# Autodesk Inventor assembly: Złożenie całości
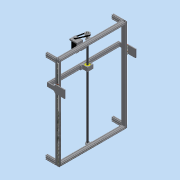
[picture p0: Inventor's stored thumbnail of the model, 180x180]
Saved by Autodesk Inventor 2018 (Build 220112000, 112)
## iProperties
Created: 2019-01-23
Part Number: Złożenie całości
Material: Ogólny
Document SubType Name: Assembly
Designer: Dawid
Author: Dawid
## Documents named in this file (24)
- E:\Frezarka_K2\INVENTOR\ZŁOŻENIA\Złożenie całości.iam
- E:\Frezarka_K2\INVENTOR\RAMA\Profil dolny długi.ipt
- E:\Frezarka_K2\INVENTOR\RAMA\Profil dolny krótki.ipt
- E:\Frezarka_K2\INVENTOR\RAMA\Profil dolny - noga.ipt
- E:\Frezarka_K2\INVENTOR\NAPĘD\Śruba trapezowa 16x4.ipt
- E:\Frezarka_K2\INVENTOR\NAPĘD\Łożysko w obudowie aluminiowej 10mm KP000.ipt
- C:\Users\Dawid\Documents\Inventor\Content Center Files\R2018\pl-PL\DIN 6926\DIN 6926 - M10 x 1,5.ipt
- E:\Frezarka_K2\INVENTOR\NAPĘD\Koło zębate 21 T5 28 2F.ipt
- E:\Frezarka_K2\INVENTOR\NAPĘD\Tuleja zaciskowo rozprężna RCK BK 80 8x15 Clampex.ipt
- C:\Users\Dawid\Documents\Inventor\Content Center Files\R2018\pl-PL\CNS 3932\CNS 3932 - M 4 x 0,7 x 6.ipt
- E:\Frezarka_K2\INVENTOR\NAPĘD\Silnik krokowy SM 60 100-4004AF - 4Nm.ipt
- E:\Frezarka_K2\INVENTOR\NAPĘD\Koło zębate 21 T5 14 2F.ipt
- E:\Frezarka_K2\INVENTOR\NAPĘD\Uchwyt silnika krokowego osi Y.ipt
- C:\Users\Dawid\Documents\Inventor\Content Center Files\R2018\pl-PL\CNS 3932\CNS 3932 - M 5 x 0,8 x 12.ipt
- E:\Frezarka_K2\INVENTOR\NAPĘD\Pas zębaty 10 T5-315.ipt
- C:\Users\Dawid\Documents\Inventor\Content Center Files\R2018\pl-PL\CNS 3932\CNS 3932 - M 5 x 0,8 x 10.ipt
- E:\Frezarka_K2\INVENTOR\NAPĘD\Nakrętka trapezowa kołnierzowa JFRM-2835TR16x4.ipt
- E:\Frezarka_K2\INVENTOR\NAPĘD\Obudowa nakrętki trapezowej fi 16.ipt
- E:\Frezarka_K2\INVENTOR\RAMA\Profil dolny posuwu osi Y.ipt
- E:\Frezarka_K2\INVENTOR\NAPĘD\Prowadnica liniowa MGN9R 900mm.ipt
- E:\Frezarka_K2\INVENTOR\NAPĘD\Wózek MGN9C.ipt
- E:\Frezarka_K2\INVENTOR\NAPĘD\Wspornik pionowy osi Y.ipt
- C:\Users\Dawid\Documents\Inventor\Content Center Files\R2018\pl-PL\CNS 3932\CNS 3932 - M 3 x 0,5 x 5.ipt
- E:\Frezarka_K2\INVENTOR\RAMA\Sklejka stołu.ipt
## Components (82 placed, 23 different names)
1. Profil dolny długi:1 — Zestawiający:1, Zestawiający:4, Równoległy:19, Równoległy:20, Zestawiający:35, Zestawiający:40, Równoległy:28, Równoległy:29, Zestawiający:41, Równoległy:30, Równoległy:31, Zestawiający:44, Równoległy:36, Równoległy:43, Równoległy:44, Równoległy:45
2. Profil dolny krótki:1 — Zestawiający:1, Zestawiający:2, Równoległy:23, Równoległy:24, Zestawiający:38, Zestawiający:61, Równoległy:49
3. Profil dolny długi:2 — Zestawiający:2, Zestawiający:3, Zestawiający:5, Zestawiający:6, Zestawiający:20, Równoległy:21, Równoległy:22, Równoległy:23, Równoległy:24, Zestawiający:39, Równoległy:26, Równoległy:27, Zestawiający:42, Równoległy:32, Równoległy:33, Zestawiający:45, Równoległy:38, Równoległy:48
4. Profil dolny krótki:2 — Zestawiający:3, Równoległy:19, Równoległy:20, Równoległy:21, Równoległy:22, Zestawiający:34, Równoległy:25, Zestawiający:36, Zestawiający:37, Równoległy:37, Równoległy:39
5. Profil dolny - noga:1 — Zestawiający:5, Zestawiający:42, Równoległy:32, Równoległy:33
6. Profil dolny - noga:2 — Zestawiający:6, Zestawiający:39, Równoległy:26, Równoległy:27
7. Profil dolny - noga:3 — Zestawiający:41, Równoległy:30, Równoległy:31
8. Profil dolny - noga:4 — Zestawiający:4, Zestawiający:40, Równoległy:28, Równoległy:29
9. Śruba trapezowa 16x4:1 — Zestawiający:8, Zestawiający:9, Zestawiający:10, Zestawiający:11, Zestawiający:12, Zestawiający:18, Zestawiający:19, Zestawiający:31
10. Łożysko w obudowie aluminiowej 10mm KP000:1 — Zestawiający:8, Zestawiający:9, Zestawiający:13, Zestawiający:20, Zestawiający:34, Zestawiający:35, Równoległy:25
11. Łożysko w obudowie aluminiowej 10mm KP000:2 — Zestawiający:10, Zestawiający:11, Zestawiający:38
12. DIN 6926 - zastąpiona przez DIN EN 1663/1666 M10:1 — Zestawiający:12, Zestawiający:13
13. Koło zębate 21 T5 28 2F:1 — Zestawiający:16, Zestawiający:17, Zestawiający:28
14. Tuleja zaciskowo rozprężna RCK BK 80 8x15 Clampex:1 — Zestawiający:16, Zestawiający:17, Zestawiający:18, Zestawiający:19, Wstaw:1, Wstaw:2, Wstaw:3, Wstaw:4, Wstaw:5, Wstaw:6
15. CNS 3932 M 4 x 6:1 — Wstaw:1
16. CNS 3932 M 4 x 6:2 — Wstaw:2
17. CNS 3932 M 4 x 6:3 — Wstaw:3
18. CNS 3932 M 4 x 6:4 — Wstaw:4
19. CNS 3932 M 4 x 6:5 — Wstaw:5
20. CNS 3932 M 4 x 6:6 — Wstaw:6
21. Silnik krokowy SM 60 100-4004AF - 4Nm:1 — Zestawiający:21, Zestawiający:22, Zestawiający:23, Zestawiający:24, Zestawiający:25, Wstaw:7, Wstaw:8, Wstaw:9, Wstaw:10
22. Koło zębate 21 T5 14 2F:1 — Zestawiający:21, Zestawiający:22, Zestawiający:29
23. Uchwyt silnika krokowego osi Y:1 — Zestawiający:23, Zestawiający:24, Zestawiający:25, Wstaw:11, Wstaw:12, Wstaw:13, Wstaw:14, Zestawiający:36, Zestawiający:37
24. CNS 3932 M 5 x 12:1 — Wstaw:7
25. CNS 3932 M 5 x 12:2 — Wstaw:8
26. CNS 3932 M 5 x 12:3 — Wstaw:9
27. CNS 3932 M 5 x 12:4 — Wstaw:10
28. Pas zębaty 10 T5-315:1 — Zestawiający:28, Zestawiający:29
29. CNS 3932 M 5 x 10:1 — Wstaw:11
30. CNS 3932 M 5 x 10:2 — Wstaw:12
31. CNS 3932 M 5 x 10:3 — Wstaw:13
32. CNS 3932 M 5 x 10:4 — Wstaw:14
33. Nakrętka trapezowa kołnierzowa JFRM-2835TR16x4:1 — Zestawiający:31, Zestawiający:32, Zestawiający:33
34. Obudowa nakrętki trapezowej fi 16:1 — Zestawiający:32, Zestawiający:33, Równoległy:18, Zestawiający:43, Równoległy:34, Równoległy:35
35. Profil dolny posuwu osi Y:1 — Równoległy:18, Zestawiający:43, Równoległy:34, Równoległy:35, Równoległy:40, Zestawiający:54, Równoległy:41, Równoległy:42, Zestawiający:58, Równoległy:46, Równoległy:47
36. Prowadnica liniowa MGN9R 900mm:1 — Zestawiający:44, Równoległy:36, Równoległy:37, Zestawiający:50, Zestawiający:51, Zestawiający:52, Zestawiający:53, Wstaw:34, Wstaw:35, Wstaw:36, Wstaw:37, Wstaw:38, Wstaw:39, Wstaw:40, Wstaw:41, Wstaw:42, Wstaw:43, Wstaw:44, Wstaw:45, Wstaw:46, Wstaw:47, Wstaw:48, Wstaw:49, Wstaw:50, Wstaw:51, Wstaw:52
37. Prowadnica liniowa MGN9R 900mm:2 — Zestawiający:45, Równoległy:38, Równoległy:39, Zestawiający:46, Zestawiający:47, Zestawiający:48, Zestawiający:49, Zestawiający:57, Wstaw:15, Wstaw:16, Wstaw:17, Wstaw:18, Wstaw:19, Wstaw:20, Wstaw:21, Wstaw:22, Wstaw:23, Wstaw:24, Wstaw:25, Wstaw:26, Wstaw:27, Wstaw:28, Wstaw:29, Wstaw:30, Wstaw:31, Wstaw:32, Wstaw:33
38. Wózek MGN9C:1 — Zestawiający:46, Zestawiający:47, Zestawiający:59
39. Wózek MGN9C:2 — Zestawiający:48, Zestawiający:49, Zestawiający:57, Zestawiający:60
40. Wózek MGN9C:3 — Zestawiający:50, Zestawiający:51, Zestawiający:55
41. Wózek MGN9C:4 — Zestawiający:52, Zestawiający:53, Równoległy:40, Zestawiający:56
42. Wspornik pionowy osi Y:1 — Zestawiający:54, Równoległy:41, Równoległy:42, Zestawiający:55, Zestawiający:56
43. Wspornik pionowy osi Y:2 — Zestawiający:58, Równoległy:46, Równoległy:47, Zestawiający:59, Zestawiający:60
44. CNS 3932 M 3 x 5:1 — Wstaw:15
45. CNS 3932 M 3 x 5:2 — Wstaw:16
46. CNS 3932 M 3 x 5:3 — Wstaw:17
47. CNS 3932 M 3 x 5:4 — Wstaw:18
48. CNS 3932 M 3 x 5:5 — Wstaw:19
49. CNS 3932 M 3 x 5:6 — Wstaw:20
50. CNS 3932 M 3 x 5:7 — Wstaw:21
51. CNS 3932 M 3 x 5:8 — Wstaw:22
52. CNS 3932 M 3 x 5:9 — Wstaw:23
53. CNS 3932 M 3 x 5:10 — Wstaw:24
54. CNS 3932 M 3 x 5:11 — Wstaw:25
55. CNS 3932 M 3 x 5:12 — Wstaw:26
56. CNS 3932 M 3 x 5:13 — Wstaw:27
57. CNS 3932 M 3 x 5:14 — Wstaw:28
58. CNS 3932 M 3 x 5:15 — Wstaw:29
59. CNS 3932 M 3 x 5:16 — Wstaw:30
60. CNS 3932 M 3 x 5:17 — Wstaw:31
61. CNS 3932 M 3 x 5:18 — Wstaw:32
62. CNS 3932 M 3 x 5:19 — Wstaw:33
63. CNS 3932 M 3 x 5:20 — Wstaw:34
64. CNS 3932 M 3 x 5:21 — Wstaw:35
65. CNS 3932 M 3 x 5:22 — Wstaw:36
66. CNS 3932 M 3 x 5:23 — Wstaw:37
67. CNS 3932 M 3 x 5:24 — Wstaw:38
68. CNS 3932 M 3 x 5:25 — Wstaw:39
69. CNS 3932 M 3 x 5:26 — Wstaw:40
70. CNS 3932 M 3 x 5:27 — Wstaw:41
71. CNS 3932 M 3 x 5:28 — Wstaw:42
72. CNS 3932 M 3 x 5:29 — Wstaw:43
73. CNS 3932 M 3 x 5:30 — Wstaw:44
74. CNS 3932 M 3 x 5:31 — Wstaw:45
75. CNS 3932 M 3 x 5:32 — Wstaw:46
76. CNS 3932 M 3 x 5:33 — Wstaw:47
77. CNS 3932 M 3 x 5:34 — Wstaw:48
78. CNS 3932 M 3 x 5:35 — Wstaw:49
79. CNS 3932 M 3 x 5:36 — Wstaw:50
80. CNS 3932 M 3 x 5:37 — Wstaw:51
81. CNS 3932 M 3 x 5:38 — Wstaw:52
82. Sklejka stołu:1 — Zestawiający:61, Równoległy:48, Równoległy:49
## Relationships (139: Mate 55, Insert 52, Flush 32)
- Zestawiający:1 [Mate]: Profil dolny długi:1 ↔ Profil dolny krótki:1
- Zestawiający:2 [Mate]: Profil dolny krótki:1 ↔ Profil dolny długi:2
- Zestawiający:3 [Mate]: Profil dolny długi:2 ↔ Profil dolny krótki:2
- Zestawiający:4 [Mate]: Profil dolny długi:1 ↔ Profil dolny - noga:4
- Zestawiający:5 [Mate]: Profil dolny długi:2 ↔ Profil dolny - noga:1
- Zestawiający:6 [Mate]: Profil dolny długi:2 ↔ Profil dolny - noga:2
- Zestawiający:8 [Mate]: Śruba trapezowa 16x4:1 ↔ Łożysko w obudowie aluminiowej 10mm KP000:1
- Zestawiający:9 [Mate]: Śruba trapezowa 16x4:1 ↔ Łożysko w obudowie aluminiowej 10mm KP000:1
- Zestawiający:10 [Mate]: Śruba trapezowa 16x4:1 ↔ Łożysko w obudowie aluminiowej 10mm KP000:2
- Zestawiający:11 [Mate] (2 mm): Śruba trapezowa 16x4:1 ↔ Łożysko w obudowie aluminiowej 10mm KP000:2
- Zestawiający:12 [Mate]: Śruba trapezowa 16x4:1 ↔ DIN 6926 - zastąpiona przez DIN EN 1663/1666 M10:1
- Zestawiający:13 [Mate]: Łożysko w obudowie aluminiowej 10mm KP000:1 ↔ DIN 6926 - zastąpiona przez DIN EN 1663/1666 M10:1
- Zestawiający:16 [Mate]: Koło zębate 21 T5 28 2F:1 ↔ Tuleja zaciskowo rozprężna RCK BK 80 8x15 Clampex:1
- Zestawiający:17 [Mate]: Koło zębate 21 T5 28 2F:1 ↔ Tuleja zaciskowo rozprężna RCK BK 80 8x15 Clampex:1
- Zestawiający:18 [Mate]: Śruba trapezowa 16x4:1 ↔ Tuleja zaciskowo rozprężna RCK BK 80 8x15 Clampex:1
- Zestawiający:19 [Mate] (2 mm): Śruba trapezowa 16x4:1 ↔ Tuleja zaciskowo rozprężna RCK BK 80 8x15 Clampex:1
- Wstaw:1 [Insert]: Tuleja zaciskowo rozprężna RCK BK 80 8x15 Clampex:1 ↔ CNS 3932 M 4 x 6:1
- Wstaw:2 [Insert]: Tuleja zaciskowo rozprężna RCK BK 80 8x15 Clampex:1 ↔ CNS 3932 M 4 x 6:2
- Wstaw:3 [Insert]: Tuleja zaciskowo rozprężna RCK BK 80 8x15 Clampex:1 ↔ CNS 3932 M 4 x 6:3
- Wstaw:4 [Insert]: Tuleja zaciskowo rozprężna RCK BK 80 8x15 Clampex:1 ↔ CNS 3932 M 4 x 6:4
- Wstaw:5 [Insert]: Tuleja zaciskowo rozprężna RCK BK 80 8x15 Clampex:1 ↔ CNS 3932 M 4 x 6:5
- Wstaw:6 [Insert]: Tuleja zaciskowo rozprężna RCK BK 80 8x15 Clampex:1 ↔ CNS 3932 M 4 x 6:6
- Zestawiający:20 [Mate] (296.5 mm): Profil dolny długi:2 ↔ Łożysko w obudowie aluminiowej 10mm KP000:1
- Zestawiający:21 [Mate]: Silnik krokowy SM 60 100-4004AF - 4Nm:1 ↔ Koło zębate 21 T5 14 2F:1
- Zestawiający:22 [Mate] (1 mm): Silnik krokowy SM 60 100-4004AF - 4Nm:1 ↔ Koło zębate 21 T5 14 2F:1
- Zestawiający:23 [Mate]: Silnik krokowy SM 60 100-4004AF - 4Nm:1 ↔ Uchwyt silnika krokowego osi Y:1
- Zestawiający:24 [Mate]: Silnik krokowy SM 60 100-4004AF - 4Nm:1 ↔ Uchwyt silnika krokowego osi Y:1
- Zestawiający:25 [Mate]: Silnik krokowy SM 60 100-4004AF - 4Nm:1 ↔ Uchwyt silnika krokowego osi Y:1
- Wstaw:7 [Insert]: Silnik krokowy SM 60 100-4004AF - 4Nm:1 ↔ CNS 3932 M 5 x 12:1
- Wstaw:8 [Insert]: Silnik krokowy SM 60 100-4004AF - 4Nm:1 ↔ CNS 3932 M 5 x 12:2
- Wstaw:9 [Insert]: Silnik krokowy SM 60 100-4004AF - 4Nm:1 ↔ CNS 3932 M 5 x 12:3
- Wstaw:10 [Insert]: Silnik krokowy SM 60 100-4004AF - 4Nm:1 ↔ CNS 3932 M 5 x 12:4
- Zestawiający:28 [Mate]: Koło zębate 21 T5 28 2F:1 ↔ Pas zębaty 10 T5-315:1
- Zestawiający:29 [Mate]: Koło zębate 21 T5 14 2F:1 ↔ Pas zębaty 10 T5-315:1
- Wstaw:11 [Insert]: Uchwyt silnika krokowego osi Y:1 ↔ CNS 3932 M 5 x 10:1
- Wstaw:12 [Insert]: Uchwyt silnika krokowego osi Y:1 ↔ CNS 3932 M 5 x 10:2
- Wstaw:13 [Insert]: Uchwyt silnika krokowego osi Y:1 ↔ CNS 3932 M 5 x 10:3
- Wstaw:14 [Insert]: Uchwyt silnika krokowego osi Y:1 ↔ CNS 3932 M 5 x 10:4
- Zestawiający:31 [Mate]: Śruba trapezowa 16x4:1 ↔ Nakrętka trapezowa kołnierzowa JFRM-2835TR16x4:1
- Zestawiający:32 [Mate]: Nakrętka trapezowa kołnierzowa JFRM-2835TR16x4:1 ↔ Obudowa nakrętki trapezowej fi 16:1
- Zestawiający:33 [Mate]: Nakrętka trapezowa kołnierzowa JFRM-2835TR16x4:1 ↔ Obudowa nakrętki trapezowej fi 16:1
- Równoległy:18 [Flush] (310 mm): Obudowa nakrętki trapezowej fi 16:1 ↔ Profil dolny posuwu osi Y:1
- Równoległy:19 [Flush]: Profil dolny długi:1 ↔ Profil dolny krótki:2
- Równoległy:20 [Flush]: Profil dolny długi:1 ↔ Profil dolny krótki:2
- Równoległy:21 [Flush]: Profil dolny długi:2 ↔ Profil dolny krótki:2
- Równoległy:22 [Flush]: Profil dolny długi:2 ↔ Profil dolny krótki:2
- Równoległy:23 [Flush]: Profil dolny krótki:1 ↔ Profil dolny długi:2
- Równoległy:24 [Flush]: Profil dolny krótki:1 ↔ Profil dolny długi:2
- Zestawiający:34 [Mate]: Profil dolny krótki:2 ↔ Łożysko w obudowie aluminiowej 10mm KP000:1
- Zestawiający:35 [Mate] (296.5 mm): Profil dolny długi:1 ↔ Łożysko w obudowie aluminiowej 10mm KP000:1
- Równoległy:25 [Flush] (2 mm): Profil dolny krótki:2 ↔ Łożysko w obudowie aluminiowej 10mm KP000:1
- Zestawiający:36 [Mate]: Profil dolny krótki:2 ↔ Uchwyt silnika krokowego osi Y:1
- Zestawiający:37 [Mate]: Profil dolny krótki:2 ↔ Uchwyt silnika krokowego osi Y:1
- Zestawiający:38 [Mate]: Profil dolny krótki:1 ↔ Łożysko w obudowie aluminiowej 10mm KP000:2
- Zestawiający:39 [Mate]: Profil dolny długi:2 ↔ Profil dolny - noga:2
- Równoległy:26 [Flush]: Profil dolny długi:2 ↔ Profil dolny - noga:2
- Równoległy:27 [Flush]: Profil dolny długi:2 ↔ Profil dolny - noga:2
- Zestawiający:40 [Mate]: Profil dolny długi:1 ↔ Profil dolny - noga:4
- Równoległy:28 [Flush]: Profil dolny długi:1 ↔ Profil dolny - noga:4
- Równoległy:29 [Flush]: Profil dolny długi:1 ↔ Profil dolny - noga:4
- Zestawiający:41 [Mate]: Profil dolny długi:1 ↔ Profil dolny - noga:3
- Równoległy:30 [Flush]: Profil dolny długi:1 ↔ Profil dolny - noga:3
- Równoległy:31 [Flush]: Profil dolny długi:1 ↔ Profil dolny - noga:3
- Zestawiający:42 [Mate]: Profil dolny długi:2 ↔ Profil dolny - noga:1
- Równoległy:32 [Flush]: Profil dolny długi:2 ↔ Profil dolny - noga:1
- Równoległy:33 [Flush]: Profil dolny długi:2 ↔ Profil dolny - noga:1
- Zestawiający:43 [Mate]: Obudowa nakrętki trapezowej fi 16:1 ↔ Profil dolny posuwu osi Y:1
- Równoległy:34 [Flush]: Obudowa nakrętki trapezowej fi 16:1 ↔ Profil dolny posuwu osi Y:1
- Równoległy:35 [Flush] (310 mm): Obudowa nakrętki trapezowej fi 16:1 ↔ Profil dolny posuwu osi Y:1
- Zestawiający:44 [Mate]: Profil dolny długi:1 ↔ Prowadnica liniowa MGN9R 900mm:1
- Równoległy:36 [Flush] (25.5 mm): Profil dolny długi:1 ↔ Prowadnica liniowa MGN9R 900mm:1
- Równoległy:37 [Flush] (25 mm): Profil dolny krótki:2 ↔ Prowadnica liniowa MGN9R 900mm:1
- Zestawiający:45 [Mate]: Profil dolny długi:2 ↔ Prowadnica liniowa MGN9R 900mm:2
- Równoległy:38 [Flush] (25.5 mm): Profil dolny długi:2 ↔ Prowadnica liniowa MGN9R 900mm:2
- Równoległy:39 [Flush] (25 mm): Profil dolny krótki:2 ↔ Prowadnica liniowa MGN9R 900mm:2
- Zestawiający:46 [Mate]: Prowadnica liniowa MGN9R 900mm:2 ↔ Wózek MGN9C:1
- Zestawiający:47 [Mate]: Prowadnica liniowa MGN9R 900mm:2 ↔ Wózek MGN9C:1
- Zestawiający:48 [Mate]: Prowadnica liniowa MGN9R 900mm:2 ↔ Wózek MGN9C:2
- Zestawiający:49 [Mate]: Prowadnica liniowa MGN9R 900mm:2 ↔ Wózek MGN9C:2
- Zestawiający:50 [Mate]: Prowadnica liniowa MGN9R 900mm:1 ↔ Wózek MGN9C:3
- Zestawiający:51 [Mate]: Prowadnica liniowa MGN9R 900mm:1 ↔ Wózek MGN9C:3
- Zestawiający:52 [Mate]: Prowadnica liniowa MGN9R 900mm:1 ↔ Wózek MGN9C:4
- Zestawiający:53 [Mate]: Prowadnica liniowa MGN9R 900mm:1 ↔ Wózek MGN9C:4
- Równoległy:40 [Flush]: Profil dolny posuwu osi Y:1 ↔ Wózek MGN9C:4
- Zestawiający:54 [Mate]: Profil dolny posuwu osi Y:1 ↔ Wspornik pionowy osi Y:1
- Równoległy:41 [Flush]: Profil dolny posuwu osi Y:1 ↔ Wspornik pionowy osi Y:1
- Równoległy:42 [Flush]: Profil dolny posuwu osi Y:1 ↔ Wspornik pionowy osi Y:1
- Zestawiający:55 [Mate]: Wózek MGN9C:3 ↔ Wspornik pionowy osi Y:1
- Zestawiający:56 [Mate]: Wózek MGN9C:4 ↔ Wspornik pionowy osi Y:1
- Równoległy:43 [Flush]: Profil dolny długi:1
- Równoległy:44 [Flush]: Profil dolny długi:1
- Równoległy:45 [Flush]: Profil dolny długi:1
- Zestawiający:57 [Mate]: Prowadnica liniowa MGN9R 900mm:2 ↔ Wózek MGN9C:2
- Zestawiający:58 [Mate]: Profil dolny posuwu osi Y:1 ↔ Wspornik pionowy osi Y:2
- Równoległy:46 [Flush]: Profil dolny posuwu osi Y:1 ↔ Wspornik pionowy osi Y:2
- Równoległy:47 [Flush]: Profil dolny posuwu osi Y:1 ↔ Wspornik pionowy osi Y:2
- Zestawiający:59 [Mate]: Wózek MGN9C:1 ↔ Wspornik pionowy osi Y:2
- Zestawiający:60 [Mate]: Wózek MGN9C:2 ↔ Wspornik pionowy osi Y:2
- Wstaw:15 [Insert]: Prowadnica liniowa MGN9R 900mm:2 ↔ CNS 3932 M 3 x 5:1
- Wstaw:16 [Insert]: Prowadnica liniowa MGN9R 900mm:2 ↔ CNS 3932 M 3 x 5:2
- Wstaw:17 [Insert]: Prowadnica liniowa MGN9R 900mm:2 ↔ CNS 3932 M 3 x 5:3
- Wstaw:18 [Insert]: Prowadnica liniowa MGN9R 900mm:2 ↔ CNS 3932 M 3 x 5:4
- Wstaw:19 [Insert]: Prowadnica liniowa MGN9R 900mm:2 ↔ CNS 3932 M 3 x 5:5
- Wstaw:20 [Insert]: Prowadnica liniowa MGN9R 900mm:2 ↔ CNS 3932 M 3 x 5:6
- Wstaw:21 [Insert]: Prowadnica liniowa MGN9R 900mm:2 ↔ CNS 3932 M 3 x 5:7
- Wstaw:22 [Insert]: Prowadnica liniowa MGN9R 900mm:2 ↔ CNS 3932 M 3 x 5:8
- Wstaw:23 [Insert]: Prowadnica liniowa MGN9R 900mm:2 ↔ CNS 3932 M 3 x 5:9
- Wstaw:24 [Insert]: Prowadnica liniowa MGN9R 900mm:2 ↔ CNS 3932 M 3 x 5:10
- Wstaw:25 [Insert]: Prowadnica liniowa MGN9R 900mm:2 ↔ CNS 3932 M 3 x 5:11
- Wstaw:26 [Insert]: Prowadnica liniowa MGN9R 900mm:2 ↔ CNS 3932 M 3 x 5:12
- Wstaw:27 [Insert]: Prowadnica liniowa MGN9R 900mm:2 ↔ CNS 3932 M 3 x 5:13
- Wstaw:28 [Insert]: Prowadnica liniowa MGN9R 900mm:2 ↔ CNS 3932 M 3 x 5:14
- Wstaw:29 [Insert]: Prowadnica liniowa MGN9R 900mm:2 ↔ CNS 3932 M 3 x 5:15
- Wstaw:30 [Insert]: Prowadnica liniowa MGN9R 900mm:2 ↔ CNS 3932 M 3 x 5:16
- Wstaw:31 [Insert]: Prowadnica liniowa MGN9R 900mm:2 ↔ CNS 3932 M 3 x 5:17
- Wstaw:32 [Insert]: Prowadnica liniowa MGN9R 900mm:2 ↔ CNS 3932 M 3 x 5:18
- Wstaw:33 [Insert]: Prowadnica liniowa MGN9R 900mm:2 ↔ CNS 3932 M 3 x 5:19
- Wstaw:34 [Insert]: Prowadnica liniowa MGN9R 900mm:1 ↔ CNS 3932 M 3 x 5:20
- Wstaw:35 [Insert]: Prowadnica liniowa MGN9R 900mm:1 ↔ CNS 3932 M 3 x 5:21
- Wstaw:36 [Insert]: Prowadnica liniowa MGN9R 900mm:1 ↔ CNS 3932 M 3 x 5:22
- Wstaw:37 [Insert]: Prowadnica liniowa MGN9R 900mm:1 ↔ CNS 3932 M 3 x 5:23
- Wstaw:38 [Insert]: Prowadnica liniowa MGN9R 900mm:1 ↔ CNS 3932 M 3 x 5:24
- Wstaw:39 [Insert]: Prowadnica liniowa MGN9R 900mm:1 ↔ CNS 3932 M 3 x 5:25
- Wstaw:40 [Insert]: Prowadnica liniowa MGN9R 900mm:1 ↔ CNS 3932 M 3 x 5:26
- Wstaw:41 [Insert]: Prowadnica liniowa MGN9R 900mm:1 ↔ CNS 3932 M 3 x 5:27
- Wstaw:42 [Insert]: Prowadnica liniowa MGN9R 900mm:1 ↔ CNS 3932 M 3 x 5:28
- Wstaw:43 [Insert]: Prowadnica liniowa MGN9R 900mm:1 ↔ CNS 3932 M 3 x 5:29
- Wstaw:44 [Insert]: Prowadnica liniowa MGN9R 900mm:1 ↔ CNS 3932 M 3 x 5:30
- Wstaw:45 [Insert]: Prowadnica liniowa MGN9R 900mm:1 ↔ CNS 3932 M 3 x 5:31
- Wstaw:46 [Insert]: Prowadnica liniowa MGN9R 900mm:1 ↔ CNS 3932 M 3 x 5:32
- Wstaw:47 [Insert]: Prowadnica liniowa MGN9R 900mm:1 ↔ CNS 3932 M 3 x 5:33
- Wstaw:48 [Insert]: Prowadnica liniowa MGN9R 900mm:1 ↔ CNS 3932 M 3 x 5:34
- Wstaw:49 [Insert]: Prowadnica liniowa MGN9R 900mm:1 ↔ CNS 3932 M 3 x 5:35
- Wstaw:50 [Insert]: Prowadnica liniowa MGN9R 900mm:1 ↔ CNS 3932 M 3 x 5:36
- Wstaw:51 [Insert]: Prowadnica liniowa MGN9R 900mm:1 ↔ CNS 3932 M 3 x 5:37
- Wstaw:52 [Insert]: Prowadnica liniowa MGN9R 900mm:1 ↔ CNS 3932 M 3 x 5:38
- Zestawiający:61 [Mate]: Profil dolny krótki:1 ↔ Sklejka stołu:1
- Równoległy:48 [Flush]: Profil dolny długi:2 ↔ Sklejka stołu:1
- Równoległy:49 [Flush]: Profil dolny krótki:1 ↔ Sklejka stołu:1
